# Autodesk Inventor assembly: LegRod
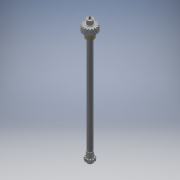
[picture p0: Inventor's stored thumbnail of the model, 180x180]
Saved by Autodesk Inventor 2019.1 (Build 231200000, 200)
## iProperties
Created: 2018-11-25
Part Number: LegRod
Material: Generisch
Document SubType Name: Assembly
Designer: JochenAlt
Author: JochenAlt
## Documents named in this file (5)
- D:\Projects\Ondine\CAD\Leg\LegRod.iam
- D:\Projects\Ondine\CAD\Leg\Stirnzahnrad21.ipt
- D:\Projects\Ondine\CAD\Spindle\SpindleWithGear.ipt
- D:\Projects\Ondine\CAD\Leg\Rod.ipt
- D:\Projects\Ondine\CAD\Leg\RodAxis.ipt
## Components (4 placed, 4 different names)
1. LegGearPinion:1 — Passend:1, Passend:2, Passend:6
2. Spindle:1 — Passend:3, Passend:4
3. Rod:1 — Passend:1, Passend:2, Passend:3, Passend:4, Passend:5
4. RodAxis:1 — Passend:5, Passend:6
## Relationships (6: Mate 6)
- Passend:1 [Mate]: LegGearPinion:1 ↔ Rod:1
- Passend:2 [Mate]: LegGearPinion:1 ↔ Rod:1
- Passend:3 [Mate]: Spindle:1 ↔ Rod:1
- Passend:4 [Mate]: Spindle:1 ↔ Rod:1
- Passend:5 [Mate]: Rod:1 ↔ RodAxis:1
- Passend:6 [Mate] (3 mm): LegGearPinion:1 ↔ RodAxis:1
